# Autodesk Inventor assembly: 300-031 (BODY SUPPORT)_MIR
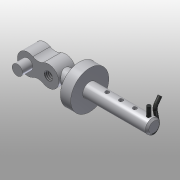
[picture p0: Inventor's stored thumbnail of the model, 180x180]
Saved by Autodesk Inventor 2015 (Build 190159000, 159)
## iProperties
Created: 2015-04-18
Part Number: 300-031 (BODY SUPPORT)_MIR
Document SubType Name: Assembly
Designer: Station9
Author: Station9
## Documents named in this file (4)
- D:\Project Archive\AD\AD-6(94.01.29)WSC2011\300-031 (BODY SUPPORT)_MIR.iam
- D:\Project Archive\AD\AD-6(94.01.29)WSC2011\500-178_MIR.ipt
- D:\Project Archive\AD\AD-6(94.01.29)WSC2011\500-177_MIR.ipt
- D:\Project Archive\AD\AD-6(94.01.29)WSC2011\500-179_MIR.ipt
## Components (3 placed, 3 different names)
1. 500-178_MIR:1 — Mate:2, Mate:1
2. 500-177_MIR:1 — Mate:2
3. 500-179_MIR:1 — Mate:1
## Relationships (2: Mate 2)
- Mate:2: 500-178_MIR:1 ↔ 500-177_MIR:1
- Mate:1: 500-178_MIR:1 ↔ 500-179_MIR:1
